# Autodesk Inventor assembly: POM_T5_01
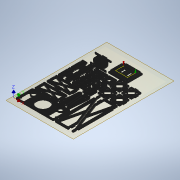
[picture p0: Inventor's stored thumbnail of the model, 180x180]
Saved by Autodesk Inventor 2020 (Build 240168000, 168)
## iProperties
Created: 2021-08-27
Part Number: POM_T5_01
Document SubType Name: Assembly
Designer: Masato
Author: Masato
## Documents named in this file (13)
- C:\Users\Masato\Documents\Inventor\CIT Brains_Inventor\OpenPlatform_ver3_0\cam\POM_T5_01.iam
- C:\Users\Masato\Documents\Inventor\CIT Brains_Inventor\OpenPlatform_ver3_0\cam\Disposable_Board.ipt
- C:\Users\Masato\Documents\Inventor\CIT Brains_Inventor\OpenPlatform_ver3_0\UpperBody\Trunk\Trunk_abdomen_spacer.ipt
- C:\Users\Masato\Documents\Inventor\CIT Brains_Inventor\OpenPlatform_ver3_0\UpperBody\Trunk\Trunk_chest_back_forth_frame.ipt
- C:\Users\Masato\Documents\Inventor\CIT Brains_Inventor\OpenPlatform_ver3_0\UpperBody\Trunk\Trunk_handle_frame.ipt
- C:\Users\Masato\Documents\Inventor\CIT Brains_Inventor\OpenPlatform_ver3_0\UpperBody\Trunk\Trunk_upper_waist_frame.ipt
- C:\Users\Masato\Documents\Inventor\CIT Brains_Inventor\OpenPlatform_ver3_0\UpperBody\Trunk\Trunk_armpit_frame.ipt
- C:\Users\Masato\Documents\Inventor\CIT Brains_Inventor\OpenPlatform_ver3_0\UpperBody\Arm\ForeArm_diagonal.ipt
- C:\Users\Masato\Documents\Inventor\CIT Brains_Inventor\OpenPlatform_ver3_0\UpperBody\Arm\UpperArm_diagonal.ipt
- C:\Users\Masato\Documents\Inventor\CIT Brains_Inventor\OpenPlatform_ver3_0\UpperBody\Head\Camera_side_frame.ipt
- C:\Users\Masato\Documents\Inventor\CIT Brains_Inventor\OpenPlatform_ver3_0\UpperBody\Head\Head_diagonal.ipt
- C:\Users\Masato\Documents\Inventor\CIT Brains_Inventor\OpenPlatform_ver3_0\UpperBody\Head\Head_horn_frame.ipt
- C:\Users\Masato\Documents\Inventor\CIT Brains_Inventor\OpenPlatform_ver3_0\UpperBody\Head\Camera_root_frame.ipt
## Components (28 placed, 12 different names)
1. Disposable_Board:1 — メイト:2, メイト:1, フラッシュ:1, フラッシュ:2, フラッシュ:3, フラッシュ:4
2. Trunk_handle_frame:1 — メイト:7, メイト:18, 正接:1, メイト:35
3. Trunk_upper_waist_frame:1 — メイト:5, フラッシュ:3, フラッシュ:4, フラッシュ:5, メイト:14, フラッシュ:7, メイト:15, メイト:16, 正接:1
4. Trunk_handle_frame:2 — メイト:9, メイト:16, メイト:17, メイト:18
5. ForeArm_diagonal:1 — メイト:10, メイト:12, フラッシュ:6, メイト:24
6. ForeArm_diagonal:2 — メイト:11, メイト:12, フラッシュ:5, メイト:14, フラッシュ:6
7. Camera_side_frame:1 — メイト:30, メイト:31, メイト:32, 正接:2
8. Head_horn_frame:1 — メイト:20, メイト:26
9. Camera_side_frame:2 — メイト:21, メイト:29, メイト:30, メイト:32, メイト:36
10. Camera_root_frame:1 — メイト:33, メイト:34, メイト:36
11. Trunk_armpit_frame:1 — メイト:4, フラッシュ:8, メイト:19, フラッシュ:10
12. Trunk_armpit_frame:2 — メイト:25
13. Trunk_armpit_frame:3 — メイト:29, 正接:2
14. Trunk_armpit_frame:4
15. Trunk_chest_back_forth_frame:1 — メイト:8, フラッシュ:7, メイト:15, メイト:17
16. Trunk_chest_back_forth_frame:2 — フラッシュ:8, メイト:19
17. Trunk_abdomen_spacer:1 — メイト:6, メイト:25, フラッシュ:10, メイト:27
18. Trunk_abdomen_spacer:2
19. Trunk_abdomen_spacer:3
20. Trunk_abdomen_spacer:4
21. Trunk_abdomen_spacer:5
22. Trunk_abdomen_spacer:6
23. Head_diagonal:1 — メイト:13, メイト:27, メイト:35
24. Head_diagonal:2 — メイト:26, メイト:28
25. UpperArm_diagonal:1 — メイト:23, メイト:28
26. UpperArm_diagonal:2 — メイト:34
27. UpperArm_diagonal:3 — メイト:24
28. UpperArm_diagonal:4
## Component patterns: (4 elements, first: Trunk_armpit_frame:1), (2 elements, first: Trunk_chest_back_forth_frame:1), (6 elements, first: Trunk_abdomen_spacer:1), (2 elements, first: Head_diagonal:1), (4 elements, first: UpperArm_diagonal:1)
## Relationships (45: Mate 34, Flush 9, Tangent 2)
- メイト:2 [Mate]: Disposable_Board:1
- メイト:1 [Mate]: Disposable_Board:1
- フラッシュ:1 [Flush]: Disposable_Board:1
- フラッシュ:2 [Flush]: Disposable_Board:1
- メイト:4 [Mate]: Trunk_armpit_frame:1
- メイト:5 [Mate]: Trunk_upper_waist_frame:1
- メイト:6 [Mate]: Trunk_abdomen_spacer:1
- メイト:7 [Mate]: Trunk_handle_frame:1
- メイト:8 [Mate]: Trunk_chest_back_forth_frame:1
- メイト:9 [Mate]: Trunk_handle_frame:2
- メイト:10 [Mate]: ForeArm_diagonal:1
- メイト:11 [Mate]: ForeArm_diagonal:2
- メイト:12 [Mate] (3 mm): ForeArm_diagonal:1 ↔ ForeArm_diagonal:2
- メイト:13 [Mate]: Head_diagonal:1
- フラッシュ:3 [Flush] (3 mm): Disposable_Board:1 ↔ Trunk_upper_waist_frame:1
- フラッシュ:4 [Flush] (3 mm): Disposable_Board:1 ↔ Trunk_upper_waist_frame:1
- フラッシュ:5 [Flush]: Trunk_upper_waist_frame:1 ↔ ForeArm_diagonal:2
- メイト:14 [Mate] (3 mm): Trunk_upper_waist_frame:1 ↔ ForeArm_diagonal:2
- フラッシュ:6 [Flush]: ForeArm_diagonal:1 ↔ ForeArm_diagonal:2
- フラッシュ:7 [Flush]: Trunk_upper_waist_frame:1 ↔ Trunk_chest_back_forth_frame:1
- メイト:15 [Mate] (3 mm): Trunk_upper_waist_frame:1 ↔ Trunk_chest_back_forth_frame:1
- メイト:16 [Mate] (3 mm): Trunk_upper_waist_frame:1 ↔ Trunk_handle_frame:2
- メイト:17 [Mate] (3 mm): Trunk_handle_frame:2 ↔ Trunk_chest_back_forth_frame:1
- メイト:18 [Mate] (3 mm): Trunk_handle_frame:1 ↔ Trunk_handle_frame:2
- 正接:1 [Tangent] (3 mm): Trunk_handle_frame:1 ↔ Trunk_upper_waist_frame:1
- フラッシュ:8 [Flush]: Trunk_armpit_frame:1 ↔ Trunk_chest_back_forth_frame:2
- メイト:19 [Mate] (3 mm): Trunk_armpit_frame:1 ↔ Trunk_chest_back_forth_frame:2
- メイト:20 [Mate]: Head_horn_frame:1
- メイト:21 [Mate]: Camera_side_frame:2
- メイト:23 [Mate]: UpperArm_diagonal:1
- メイト:24 [Mate] (3 mm): ForeArm_diagonal:1 ↔ UpperArm_diagonal:3
- メイト:25 [Mate] (2.5 mm): Trunk_armpit_frame:2 ↔ Trunk_abdomen_spacer:1
- フラッシュ:10 [Flush]: Trunk_armpit_frame:1 ↔ Trunk_abdomen_spacer:1
- メイト:26 [Mate] (2.5 mm): Head_horn_frame:1 ↔ Head_diagonal:2
- メイト:27 [Mate] (2.5 mm): Trunk_abdomen_spacer:1 ↔ Head_diagonal:1
- メイト:28 [Mate] (2.5 mm): Head_diagonal:2 ↔ UpperArm_diagonal:1
- メイト:29 [Mate] (2.5 mm): Camera_side_frame:2 ↔ Trunk_armpit_frame:3
- メイト:30 [Mate] (-43 mm): Camera_side_frame:1 ↔ Camera_side_frame:2
- メイト:31 [Mate]: Camera_side_frame:1
- メイト:32 [Mate] (3 mm): Camera_side_frame:1 ↔ Camera_side_frame:2
- 正接:2 [Tangent]: Camera_side_frame:1 ↔ Trunk_armpit_frame:3
- メイト:33 [Mate]: Camera_root_frame:1
- メイト:34 [Mate] (3 mm): Camera_root_frame:1 ↔ UpperArm_diagonal:2
- メイト:35 [Mate] (2.5 mm): Trunk_handle_frame:1 ↔ Head_diagonal:1
- メイト:36 [Mate] (2.5 mm): Camera_side_frame:2 ↔ Camera_root_frame:1
